# Autodesk Inventor assembly: DroneV01
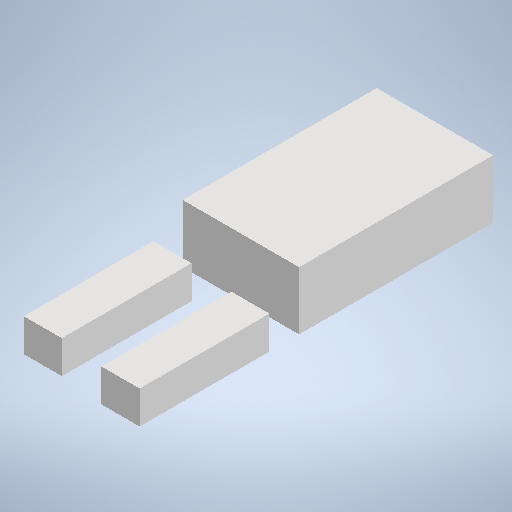
[picture p0: Inventor's stored thumbnail of the model, 512x512]
Saved by Autodesk Inventor 2025 (Build 290162000, 162)
## iProperties
Created: 2024-08-30
Part Number: DroneV01
Document SubType Name: Assembly
Designer: Cupri
Author: Cupri
## Documents named in this file (3)
- C:\Users\Cupri\OneDrive - University of South Carolina\Classes\Fall 24\Aircraft-Design-USC-Fall24\Aircraft-Design-USC-Fall24\Design\DroneV01.iam
- C:\Users\Cupri\OneDrive - University of South Carolina\Classes\Fall 24\Aircraft-Design-USC-Fall24\Aircraft-Design-USC-Fall24\Design\PlaceHoders\Battery.ipt
- C:\Users\Cupri\OneDrive - University of South Carolina\Classes\Fall 24\Aircraft-Design-USC-Fall24\Aircraft-Design-USC-Fall24\Design\PlaceHoders\SensorSuite.ipt
## Components (3 placed, 2 different names)
1. Battery:1 — Flush:2
2. Battery:2 — Flush:1, Flush:3
3. SensorSuite:1 — Flush:1, Flush:2, Flush:3
## Relationships (3: Flush 3)
- Flush:1: Battery:2 ↔ SensorSuite:1
- Flush:2: Battery:1 ↔ SensorSuite:1
- Flush:3: Battery:2 ↔ SensorSuite:1
